# Autodesk Inventor assembly: 부피 구하기4
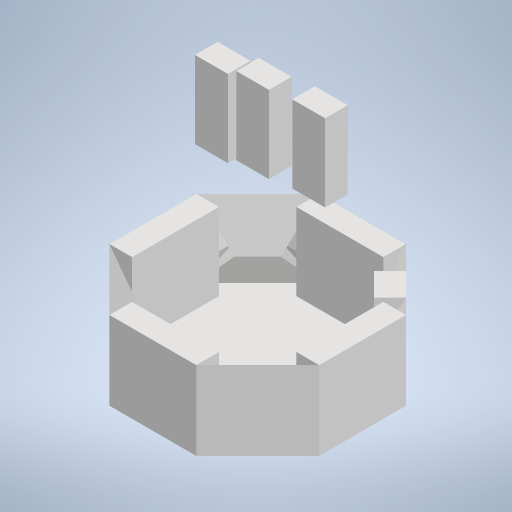
[picture p0: Inventor's stored thumbnail of the model, 512x512]
Saved by Autodesk Inventor 2024 (Build 280153000, 153)
## iProperties
Created: 2023-06-27
Part Number: 부피 구하기4
Document SubType Name: Assembly
Designer: jsw
Author: jsw
## Documents named in this file (4)
- C:\승원\co-op\OV-PAM\OV-PAM_modeling\부피 구하기4.iam
- C:\승원\co-op\OV-PAM\OV-PAM_modeling\부피 구하기2.ipt
- C:\승원\co-op\OV-PAM\OV-PAM_modeling\부피 구하기3.ipt
- C:\승원\co-op\OV-PAM\OV-PAM_modeling\부피 구하기6.ipt
## Components (9 placed, 3 different names)
1. 부피 구하기2:1 — 메이트:1, 메이트:2, 메이트:3, 메이트:4, 메이트:5, 메이트:6, 메이트:7, 메이트:8, 메이트:9, 메이트:10, 메이트:11, 메이트:12, 메이트:13, 메이트:14
2. 부피 구하기3:1 — 메이트:1, 메이트:2, 메이트:3
3. 부피 구하기3:2 — 메이트:10, 메이트:11, 메이트:12
4. 부피 구하기3:3 — 메이트:7, 메이트:8, 메이트:9
5. 부피 구하기3:4 — 메이트:4, 메이트:5, 메이트:6
6. 부피 구하기6:1
7. 부피 구하기6:2
8. 부피 구하기6:3
9. 부피 구하기6:4 — 메이트:13, 메이트:14
## Relationships (14: Mate 14)
- 메이트:1 [Mate]: 부피 구하기2:1 ↔ 부피 구하기3:1
- 메이트:2 [Mate]: 부피 구하기2:1 ↔ 부피 구하기3:1
- 메이트:3 [Mate]: 부피 구하기2:1 ↔ 부피 구하기3:1
- 메이트:4 [Mate]: 부피 구하기2:1 ↔ 부피 구하기3:4
- 메이트:5 [Mate]: 부피 구하기2:1 ↔ 부피 구하기3:4
- 메이트:6 [Mate]: 부피 구하기2:1 ↔ 부피 구하기3:4
- 메이트:7 [Mate]: 부피 구하기2:1 ↔ 부피 구하기3:3
- 메이트:8 [Mate]: 부피 구하기2:1 ↔ 부피 구하기3:3
- 메이트:9 [Mate]: 부피 구하기2:1 ↔ 부피 구하기3:3
- 메이트:10 [Mate]: 부피 구하기2:1 ↔ 부피 구하기3:2
- 메이트:11 [Mate]: 부피 구하기2:1 ↔ 부피 구하기3:2
- 메이트:12 [Mate]: 부피 구하기2:1 ↔ 부피 구하기3:2
- 메이트:13 [Mate]: 부피 구하기2:1 ↔ 부피 구하기6:4
- 메이트:14 [Mate]: 부피 구하기2:1 ↔ 부피 구하기6:4
